# Autodesk Inventor assembly: subsystem_2
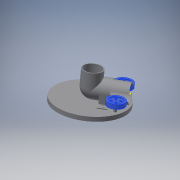
[picture p0: Inventor's stored thumbnail of the model, 180x180]
Saved by Autodesk Inventor 2019 (Build 230136000, 136)
## iProperties
Created: 2020-02-28
Part Number: subsystem_2
Document SubType Name: Assembly
Designer: Jayadev
Author: Jayadev
## Documents named in this file (10)
- G:\Inventor 2019\subsystem_2.iam
- G:\Inventor 2019\subsystem_2_clamp.ipt
- G:\Inventor 2019\subsystem_2_disc.ipt
- G:\Inventor 2019\subsystem_2_joint.ipt
- G:\Inventor 2019\subsystem_2_bent_pipe.iam.ipt
- G:\Inventor 2019\subsystem_2_disc_support_rod.ipt
- G:\Inventor 2019\subsystem_2_roller_wheels.ipt
- G:\Inventor 2019\subsystem_2_roller_wheels_disc_rod.ipt
- G:\Inventor 2019\subsystem_2_motor.ipt
- subsystem_2_bent_pipe.iam
## Components (12 placed, 8 different names)
1. subsystem_2_disc:1 — Mate:1, Mate:2, Mate:3, Mate:4, Mate:5, Mate:7, Mate:8, Flush:3, Mate:12, Mate:13, Flush:7, Flush:8, Mate:16, Mate:17
2. subsystem_2_clamp:1 — Mate:1, Mate:2, Mate:3, Flush:1, Flush:2, Mate:6
3. subsystem_2_joint:1 — Mate:5, Flush:2
4. subsystem_2_joint:2 — Mate:4, Flush:1
5. subsystem_2_bent_pipe.iam:1 — Mate:6, Mate:7
6. subsystem_2_disc_support_rod:1 — Mate:8, Flush:3
7. subsystem_2_roller_wheels:1 — Mate:10, Flush:5
8. subsystem_2_roller_wheels:2 — Mate:11, Flush:6
9. subsystem_2_roller_wheels_disc_rod:1 — Mate:10, Flush:5, Mate:12, Flush:7, Mate:14
10. subsystem_2_roller_wheels_disc_rod:2 — Mate:11, Flush:6, Mate:13, Flush:8, Mate:15
11. subsystem_2_motor:1 — Mate:14, Mate:16
12. subsystem_2_motor:2 — Mate:15, Mate:17
## Relationships (23: Mate 16, Flush 7)
- Mate:1: subsystem_2_disc:1 ↔ subsystem_2_clamp:1
- Mate:2: subsystem_2_disc:1 ↔ subsystem_2_clamp:1
- Mate:3: subsystem_2_disc:1 ↔ subsystem_2_clamp:1
- Mate:4: subsystem_2_disc:1 ↔ subsystem_2_joint:2
- Flush:1: subsystem_2_clamp:1 ↔ subsystem_2_joint:2
- Mate:5: subsystem_2_disc:1 ↔ subsystem_2_joint:1
- Flush:2: subsystem_2_clamp:1 ↔ subsystem_2_joint:1
- Mate:6: subsystem_2_clamp:1 ↔ subsystem_2_bent_pipe.iam:1
- Mate:7: subsystem_2_disc:1 ↔ subsystem_2_bent_pipe.iam:1
- Mate:8: subsystem_2_disc:1 ↔ subsystem_2_disc_support_rod:1
- Flush:3: subsystem_2_disc:1 ↔ subsystem_2_disc_support_rod:1
- Mate:10: subsystem_2_roller_wheels:1 ↔ subsystem_2_roller_wheels_disc_rod:1
- Flush:5: subsystem_2_roller_wheels:1 ↔ subsystem_2_roller_wheels_disc_rod:1
- Mate:11: subsystem_2_roller_wheels:2 ↔ subsystem_2_roller_wheels_disc_rod:2
- Flush:6: subsystem_2_roller_wheels:2 ↔ subsystem_2_roller_wheels_disc_rod:2
- Mate:12: subsystem_2_disc:1 ↔ subsystem_2_roller_wheels_disc_rod:1
- Mate:13: subsystem_2_disc:1 ↔ subsystem_2_roller_wheels_disc_rod:2
- Flush:7: subsystem_2_disc:1 ↔ subsystem_2_roller_wheels_disc_rod:1
- Flush:8: subsystem_2_disc:1 ↔ subsystem_2_roller_wheels_disc_rod:2
- Mate:14: subsystem_2_roller_wheels_disc_rod:1 ↔ subsystem_2_motor:1
- Mate:15: subsystem_2_roller_wheels_disc_rod:2 ↔ subsystem_2_motor:2
- Mate:16: subsystem_2_disc:1 ↔ subsystem_2_motor:1
- Mate:17: subsystem_2_disc:1 ↔ subsystem_2_motor:2
